# Autodesk Inventor assembly: Front Left Foot
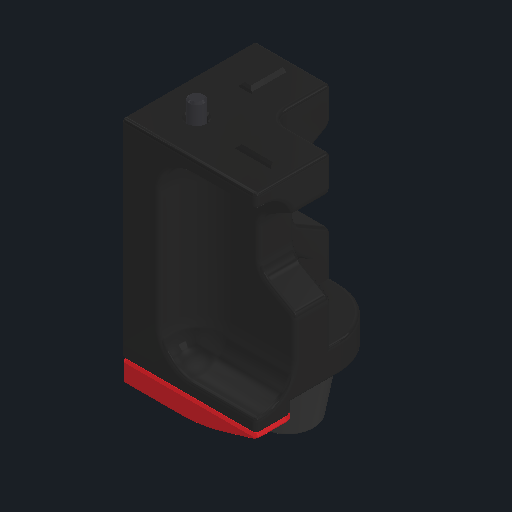
[picture p0: Inventor's stored thumbnail of the model, 512x512]
Saved by Autodesk Inventor 2025.1 (Build 291241020, 241B)
## iProperties
Created: 2025-05-09
Part Number: Front Left Foot
Document SubType Name: Assembly
Designer: AdminForWorker
Title: Front Left Foot
Author: AdminForWorker
## Documents named in this file (7)
- C:\Users\Joshua Eah\Documents\Voron 0.2\CAD\Master Assembly\Front Left Foot.iam
- C:\Users\Joshua Eah\Documents\Voron 0.2\CAD\Master Assembly\Printed Parts (23).iam
- C:\Users\Joshua Eah\Documents\Voron 0.2\CAD\Master Assembly\Rubber Feet.iam
- C:\Users\Joshua Eah\Documents\Voron 0.2\CAD\Master Assembly\Hardware\M3 Threaded Insert.ipt
- C:\Users\Joshua Eah\Documents\Voron 0.2\CAD\Master Assembly\Hardware\M2x10 Self Tapper.ipt
- C:\Users\Joshua Eah\Documents\Voron 0.2\CAD\Master Assembly\Hardware\M3x40 BHCS.ipt
- C:\Users\Joshua Eah\Documents\Voron 0.2\CAD\Master Assembly\Hardware\M3x10 BHCS.ipt
## Components (7 placed, 6 different names)
1. Printed Parts (23):1 [sub-assembly] — Insert:1, Insert:2
2. Rubber Feet:1 [sub-assembly]
3. M3 Threaded Insert (1) (2):1
4. M2x10 Self Tapper:1 — Insert:1
5. M2x10 Self Tapper:2 — Insert:2
6. M3x40 BHCS:1
7. M3x10 BHCS:1
## Relationships (2: Insert 2)
- Insert:1: Printed Parts (23):1 ↔ M2x10 Self Tapper:1
- Insert:2: Printed Parts (23):1 ↔ M2x10 Self Tapper:2
